# Autodesk Inventor assembly: Mesa
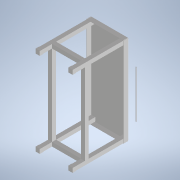
[picture p0: Inventor's stored thumbnail of the model, 180x180]
Saved by Autodesk Inventor 2021 (Build 250183000, 183)
## iProperties
Created: 2021-06-02
Part Number: Mesa
Document SubType Name: Assembly
Designer: Nelson
Author: Nelson
## Documents named in this file (6)
- D:\Nelson\Documentos\Inventor\PrensaHidraulica_Automatizada\Mesa.iam
- D:\Nelson\Documentos\Inventor\PrensaHidraulica_Automatizada\Mesa_tablero.ipt
- D:\Nelson\Documentos\Inventor\PrensaHidraulica_Automatizada\Mesa_pata.ipt
- D:\Nelson\Documentos\Inventor\PrensaHidraulica_Automatizada\Mesa_base1.ipt
- D:\Nelson\Documentos\Inventor\PrensaHidraulica_Automatizada\Mesa_base2.ipt
- D:\Nelson\Documentos\Inventor\PrensaHidraulica_Automatizada\Barra_5-8_950.ipt
## Components (10 placed, 5 different names)
1. Mesa_tablero:1 — Mate:1, Mate:2, Mate:3, Mate:4, Mate:5, Mate:6, Mate:7, Mate:8, Mate:9, Mate:10, Mate:11, Mate:12
2. Mesa_pata:1 — Mate:1, Mate:2, Mate:3, Mate:14, Flush:3
3. Mesa_pata:2 — Mate:4, Mate:5, Mate:6, Mate:13, Flush:2, Mate:15, Flush:5, Flush:6
4. Mesa_pata:3 — Mate:7, Mate:8, Mate:9, Flush:1, Flush:8
5. Mesa_pata:4 — Mate:10, Mate:11, Mate:12, Flush:4, Mate:16, Flush:7
6. Mesa_base1:1 — Mate:13, Flush:1, Flush:2
7. Mesa_base1:2 — Mate:14, Flush:3, Flush:4
8. Mesa_base2:1 — Mate:15, Flush:5, Flush:6
9. Mesa_base2:2 — Mate:16, Flush:7, Flush:8
10. Barra_5-8_950:1
## Relationships (24: Mate 16, Flush 8)
- Mate:1: Mesa_tablero:1 ↔ Mesa_pata:1
- Mate:2: Mesa_tablero:1 ↔ Mesa_pata:1
- Mate:3: Mesa_tablero:1 ↔ Mesa_pata:1
- Mate:4: Mesa_tablero:1 ↔ Mesa_pata:2
- Mate:5: Mesa_tablero:1 ↔ Mesa_pata:2
- Mate:6: Mesa_tablero:1 ↔ Mesa_pata:2
- Mate:7: Mesa_tablero:1 ↔ Mesa_pata:3
- Mate:8: Mesa_tablero:1 ↔ Mesa_pata:3
- Mate:9: Mesa_tablero:1 ↔ Mesa_pata:3
- Mate:10: Mesa_tablero:1 ↔ Mesa_pata:4
- Mate:11: Mesa_tablero:1 ↔ Mesa_pata:4
- Mate:12: Mesa_tablero:1 ↔ Mesa_pata:4
- Mate:13: Mesa_pata:2 ↔ Mesa_base1:1
- Flush:1: Mesa_pata:3 ↔ Mesa_base1:1
- Flush:2 (250 mm): Mesa_pata:2 ↔ Mesa_base1:1
- Mate:14: Mesa_pata:1 ↔ Mesa_base1:2
- Flush:3: Mesa_pata:1 ↔ Mesa_base1:2
- Flush:4 (250 mm): Mesa_pata:4 ↔ Mesa_base1:2
- Mate:15: Mesa_pata:2 ↔ Mesa_base2:1
- Flush:5: Mesa_pata:2 ↔ Mesa_base2:1
- Flush:6 (250 mm): Mesa_pata:2 ↔ Mesa_base2:1
- Mate:16: Mesa_pata:4 ↔ Mesa_base2:2
- Flush:7: Mesa_pata:4 ↔ Mesa_base2:2
- Flush:8 (250 mm): Mesa_pata:3 ↔ Mesa_base2:2
